# Autodesk Inventor assembly: sb
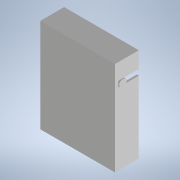
[picture p0: Inventor's stored thumbnail of the model, 180x180]
Saved by Autodesk Inventor 2022 (Build 260153000, 153)
## iProperties
Created: 2025-06-23
Part Number: sb
Document SubType Name: Assembly
Designer: korsh524
Author: korsh524
## Documents named in this file (3)
- C:\git\Olymp20205Smena\Dezign\Stemborad\sb.iam
- C:\git\Olymp20205Smena\Dezign\Stemborad\Stemboard.ipt
- C:\git\Olymp20205Smena\Dezign\Stemborad\btn.ipt
## Components (2 placed, 2 different names)
1. Stemboard:1 — Заподлицо:1
2. btn:1 — Заподлицо:1
## Relationships (1: Flush 1)
- Заподлицо:1 [Flush]: Stemboard:1 ↔ btn:1
